# Autodesk Inventor assembly: assembly
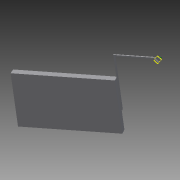
[picture p0: Inventor's stored thumbnail of the model, 180x180]
Saved by Autodesk Inventor 2014 (Build 180170000, 170)
## iProperties
Created: 2014-03-21
Part Number: assembly
Document SubType Name: Assembly
Designer: joe_000
Author: joe_000
## Documents named in this file (6)
- C:\dev\camera-multitouch\mounting-bracket\assembly.iam
- C:\dev\camera-multitouch\mounting-bracket\tv.ipt
- C:\dev\camera-multitouch\mounting-bracket\arm-vertical.ipt
- C:\dev\camera-multitouch\mounting-bracket\arm-horizontal.ipt
- C:\dev\camera-multitouch\mounting-bracket\camera.ipt
- C:\dev\camera-multitouch\mounting-bracket\cameraMount.ipt
## Components (5 placed, 5 different names)
1. tv:1 — Insert:1, Insert:2, Mate:2
2. arm-vertical:1 — Insert:1, Insert:2, Flush:1, Flush:2, Mate:1
3. arm-horizontal:1 — Flush:1, Flush:2, Mate:1, Mate:3, Mate:4, Flush:3
4. camera:1 — Mate:2, Mate:5
5. cameraMount:1 — Mate:3, Mate:4, Mate:5, Flush:3
## Relationships (10: Mate 5, Flush 3, Insert 2)
- Insert:1: tv:1 ↔ arm-vertical:1
- Insert:2: tv:1 ↔ arm-vertical:1
- Flush:1: arm-vertical:1 ↔ arm-horizontal:1
- Flush:2: arm-vertical:1 ↔ arm-horizontal:1
- Mate:1: arm-vertical:1 ↔ arm-horizontal:1
- Mate:2 (-31.75 mm): tv:1 ↔ camera:1
- Mate:3: arm-horizontal:1 ↔ cameraMount:1
- Mate:4: arm-horizontal:1 ↔ cameraMount:1
- Mate:5: camera:1 ↔ cameraMount:1
- Flush:3: arm-horizontal:1 ↔ cameraMount:1
## Named parameters: cameraLensHeight = 31.75 mm
